# Autodesk Inventor assembly: left_lower_arm_thick
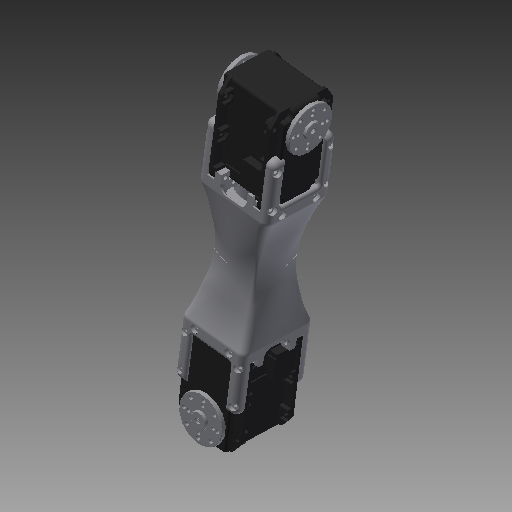
[picture p0: Inventor's stored thumbnail of the model, 512x512]
Saved by Autodesk Inventor 2019 (Build 230136000, 136)
## iProperties
Created: 2015-08-06
Part Number: left_lower_arm_thick
Document SubType Name: Assembly
Designer: 4wieser
Mass: 192.147 g
Surface Area: 567.278 cm^2
Volume: 192.147 cm^3
Density: 1 g/cm^3
Author: 4wieser
## Documents named in this file (4)
- Z:\nico\arms\left_lower_arm_thick.iam
- Z:\nico\motors\Mx64\Mx64_with_horn_and_bearing_MIR.iam
- Z:\nico\motors\Mx64\Mx64_with_horn_and_bearing_MIR1.iam
- Z:\nico\arms\upper_arm.iam
## Components (3 placed, 3 different names)
1. Mx64_with_horn_and_bearing_MIR:1 [sub-assembly] — Mate:1, Mate:2, Mate:3
2. Mx64_with_horn_and_bearing_MIR1:1 [sub-assembly] — Mate:4, Mate:5, Mate:6
3. upper_arm:1 [sub-assembly] — Mate:1, Mate:2, Mate:3, Mate:4, Mate:5, Mate:6
## Relationships (6: Mate 6)
- Mate:1: Mx64_with_horn_and_bearing_MIR:1 ↔ upper_arm:1
- Mate:2: Mx64_with_horn_and_bearing_MIR:1 ↔ upper_arm:1
- Mate:3: Mx64_with_horn_and_bearing_MIR:1 ↔ upper_arm:1
- Mate:4: Mx64_with_horn_and_bearing_MIR1:1 ↔ upper_arm:1
- Mate:5: Mx64_with_horn_and_bearing_MIR1:1 ↔ upper_arm:1
- Mate:6: Mx64_with_horn_and_bearing_MIR1:1 ↔ upper_arm:1
